# Autodesk Inventor assembly: VersaPlanetary 3 to 1 gear stage no ring
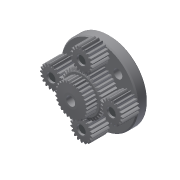
[picture p0: Inventor's stored thumbnail of the model, 180x180]
Saved by Autodesk Inventor 2013 (Build 170138000, 138)
## iProperties
Created: 2013-12-16
Part Number: VersaPlanetary 3 to 1 gear stage no ring
Document SubType Name: Assembly
Designer: Nemo
Author: Nemo
## Documents named in this file (5)
- H:\Nemo\Documents\Robotics\COTS Parts\VersaPlanetary\Components\Gear Stages\VersaPlanetary 3 to 1 gear stage no ring.iam
- H:\Nemo\Documents\Robotics\COTS Parts\VersaPlanetary\Components\Gear Stages\VersaPlanetary GR3 stage plate.ipt
- H:\Nemo\Documents\Robotics\COTS Parts\VersaPlanetary\Components\Gear Stages\VersaPlanetary GR3 stage planet axle.ipt
- H:\Nemo\Documents\Robotics\COTS Parts\VersaPlanetary\Components\Gear Stages\VersaPlanetary GR3 stage planet gear.ipt
- H:\Nemo\Documents\Robotics\COTS Parts\VersaPlanetary\Components\Gear Stages\VersaPlanetary GR3 stage sun gear.ipt
## Components (10 placed, 4 different names)
1. VersaPlanetary GR3 stage plate:1 — Mate:1, Insert:1, Insert:2, Mate:2
2. VersaPlanetary GR3 stage sun gear:1 — Mate:1, Mate:2
3. VersaPlanetary GR3 stage planet axle:1 — Insert:1
4. VersaPlanetary GR3 stage planet gear:1 — Insert:2
5. VersaPlanetary GR3 stage planet axle:2
6. VersaPlanetary GR3 stage planet gear:2
7. VersaPlanetary GR3 stage planet axle:3
8. VersaPlanetary GR3 stage planet gear:3
9. VersaPlanetary GR3 stage planet axle:4
10. VersaPlanetary GR3 stage planet gear:4
## Component patterns: (4 elements, first: VersaPlanetary GR3 stage planet axle:1 + VersaPlanetary GR3 stage planet gear:1)
## Relationships (4: Mate 2, Insert 2)
- Mate:1: VersaPlanetary GR3 stage plate:1 ↔ VersaPlanetary GR3 stage sun gear:1
- Insert:1: VersaPlanetary GR3 stage plate:1 ↔ VersaPlanetary GR3 stage planet axle:1
- Insert:2: VersaPlanetary GR3 stage plate:1 ↔ VersaPlanetary GR3 stage planet gear:1
- Mate:2: VersaPlanetary GR3 stage plate:1 ↔ VersaPlanetary GR3 stage sun gear:1
